# Autodesk Inventor assembly: MotionBaseGeneric
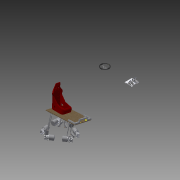
[picture p0: Inventor's stored thumbnail of the model, 180x180]
Saved by Autodesk Inventor 2015 SP1 (Build 190203100, 203)
## iProperties
Created: 2016-02-02
Part Number: MotionBaseGeneric
Document SubType Name: Assembly
Designer: tuttlem
Author: tuttlem
## Documents named in this file (17)
- C:\Users\jonesdm\Desktop\MotionBase\CAD\MotionBaseCAD\MotionBaseGeneric.iam
- C:\Users\jonesdm\Desktop\MotionBase\CAD\MotionBaseCAD\Platform.ipt
- C:\Users\jonesdm\Desktop\MotionBase\CAD\MotionBaseCAD\BasePlatform.ipt
- C:\Users\jonesdm\Desktop\MotionBase\CAD\MotionBaseCAD\Rod.ipt
- C:\Users\jonesdm\Desktop\MotionBase\CAD\MotionBaseCAD\Rod_MIR.ipt
- C:\Users\jonesdm\Desktop\MotionBase\CAD\MotionBaseCAD\arm.ipt
- C:\Users\jonesdm\Desktop\MotionBase\CAD\MotionBaseCAD\Bearing.ipt
- C:\Users\jonesdm\Desktop\MotionBase\CAD\MotionBaseCAD\siege.ipt
- C:\Users\jonesdm\Desktop\MotionBase\CAD\MotionBaseCAD\Sparco Volante wheel.ipt
- C:\Users\jonesdm\Desktop\MotionBase\CAD\MotionBaseCAD\TopPlatform.ipt
- C:\Users\jonesdm\Documents\Inventor\00 - Pedalier CSP V2.iam
- C:\Users\jonesdm\Desktop\MotionBase\CAD\MotionBaseCAD\Side Rail.ipt
- C:\Users\jonesdm\Desktop\MotionBase\CAD\MotionBaseCAD\Front Rail.ipt
- C:\Users\jonesdm\Desktop\MotionBase\CAD\MotionBaseCAD\Imported Components\WGA-50M-080-H1\WGA-50M-080-H1.ipt
- C:\Users\jonesdm\Documents\Motor4.ipt
- C:\Users\jonesdm\Desktop\MotionBase\CAD\MotionBaseCAD\GearShaft.ipt
- C:\Users\jonesdm\Desktop\MotionBase\CAD\MotionBaseCAD\Triangle.ipt
## Components (53 placed, 16 different names)
1. Platform:1 — Insert:3, Insert:5, Mate:1, Flush:7, Mate:2, Flush:8, Mate:3, Mate:4, Mate:5, Flush:9, Wood To Metal, Wood To Back, Mate:66
2. seat — Seat To Wood, Seat To Back, Seat Centered, Angle:9, Mate:72
3. Sparco Volante wheel:1
4. TopPlatform:1 — Wood To Metal, Wood To Back, Angle:8, Seat To Left, Seat To Wood, Seat To Back, Seat Centered, Mate:75, Mate:76, Flush:24, Flush:25, Flush:26, Flush:27, Mate:77, Flush:29, Flush:30, Mate:78, Flush:31, Flush:32
5. Side Rail:1 — Mate:75, Flush:24, Flush:26
6. Side Rail:2 — Mate:76, Flush:25, Flush:27
7. Front Rail:1 — Mate:77, Flush:29, Flush:30
8. Front Rail:2 — Mate:78, Flush:31, Flush:32
9. 00 - Pedalier CSP V2:2 [sub-assembly]
10. GearShaft:2 — Mate:109, Flush:40, Flush:45, Mate:148, Mate:149, Flush:55
11. GearShaft:4 — Mate:111, Flush:42, Flush:45, Mate:146, Mate:147, Flush:54
12. BasePlatform:2
13. GearShaft:8 — Mate:152, Mate:153, Flush:57
14. GearShaft:9 — Mate:154, Mate:155, Flush:58
15. GearShaft:10 — Mate:156, Mate:157, Flush:59
16. GearShaft:11 — Mate:150, Mate:151, Flush:56
17. Triangle:1 — Angle:18, Mate:137, Mate:138, Mate:139, Mate:140, Mate:141, Mate:142
18. Motor4:11 — Flush:52, Mate:129, Angle:16, Angle:17, Symmetry:3
19. Motor4:10 — Flush:52, Symmetry:3
20. Motor4:9 — Flush:53, Mate:130, Angle:16, Symmetry:2
21. Motor4:8 — Flush:53, Symmetry:2
22. Motor4:7 — Mate:96, Angle:17, Symmetry:4
23. Motor4:1 — Mate:79, Angle:10, Mate:80, Mate:91, Symmetry:4
24. Rod_MIR:1 — Flush:1, Tangent:1, Mate:100, Mate:101
25. Rod_MIR:2 — Mate:98, Mate:99
26. Rod_MIR:3 — Mate:28
27. Rod_MIR:4 — Mate:29
28. Rod_MIR:5 — Mate:97
29. Rod_MIR:6 — Mate:32
30. Rod:1 — Flush:1, Tangent:1, Insert:3
31. Rod:2 — Insert:5
32. Rod:3 — Mate:1, Flush:7
33. Rod:4 — Mate:2, Flush:8
34. Rod:5 — Mate:3, Mate:4
35. Rod:6 — Mate:5, Flush:9
36. arm:1 — Mate:146, Mate:147, Flush:54, Mate:162, Flush:64
37. arm:8 — Mate:156, Mate:157, Flush:59, Mate:159, Flush:61
38. arm:9 — Mate:150, Mate:151, Flush:56, Mate:160, Flush:62
39. arm:10 — Mate:154, Mate:155, Flush:58, Mate:158, Flush:60
40. arm:11 — Mate:148, Mate:149, Flush:55, Mate:161, Flush:63
41. arm:12 — Mate:152, Mate:153, Flush:57, Mate:163, Flush:65
42. Bearing:2 — Mate:100, Mate:101, Mate:162, Flush:64
43. Bearing:3 — Mate:97, Mate:159, Flush:61
44. Bearing:4 — Mate:32, Mate:158, Flush:60
45. Bearing:5 — Mate:29, Mate:161, Flush:63
46. Bearing:6 — Mate:28, Mate:160, Flush:62
47. Bearing:1 — Mate:98, Mate:99, Mate:163, Flush:65
48. WGA-50M-080-H1:8 — Mate:136
49. WGA-50M-080-H1:9 — Mate:135
50. WGA-50M-080-H1:10 — Mate:134
51. WGA-50M-080-H1:11 — Mate:133
52. WGA-50M-080-H1:1 — Mate:79, Angle:10, Mate:80, Mate:109, Flush:40, Mate:114, Mate:132
53. WGA-50M-080-H1:7 — Mate:111, Flush:42, Mate:114, Mate:131
## Relationships (147: Mate 80, Flush 44, Angle 12, Tangent 6, Symmetry 3, Insert 2)
- Flush:1: Rod_MIR:1 ↔ Rod:1
- Tangent:1: Rod_MIR:1 ↔ Rod:1
- [Flush]: Rod_MIR:2 ↔ Rod:2
- [Tangent]: Rod_MIR:2 ↔ Rod:2
- Insert:3: Platform:1 ↔ Rod:1
- Insert:5: Platform:1 ↔ Rod:2
- [Flush]: Rod_MIR:3 ↔ Rod:3
- [Tangent]: Rod_MIR:3 ↔ Rod:3
- [Flush]: Rod_MIR:4 ↔ Rod:4
- [Tangent]: Rod_MIR:4 ↔ Rod:4
- [Flush]: Rod_MIR:5 ↔ Rod:5
- [Tangent]: Rod_MIR:5 ↔ Rod:5
- [Flush]: Rod_MIR:6 ↔ Rod:6
- [Tangent]: Rod_MIR:6 ↔ Rod:6
- Mate:1: Platform:1 ↔ Rod:3
- Flush:7: Platform:1 ↔ Rod:3
- Mate:2: Platform:1 ↔ Rod:4
- Flush:8: Platform:1 ↔ Rod:4
- Mate:3: Platform:1 ↔ Rod:5
- Mate:4: Platform:1 ↔ Rod:5
- Mate:5: Platform:1 ↔ Rod:6
- Flush:9: Platform:1 ↔ Rod:6
- Flush:10 (25.4 mm)
- Mate:28: Rod_MIR:3 ↔ Bearing:6
- Mate:29: Rod_MIR:4 ↔ Bearing:5
- Mate:32: Rod_MIR:6 ↔ Bearing:4
- Angle:7 (0 deg)
- Wood To Metal [Mate]: Platform:1 ↔ TopPlatform:1
- Wood To Back [Flush] (-101.6 mm): Platform:1 ↔ TopPlatform:1
- Mate:66: Platform:1
- Angle:8 (0 deg): TopPlatform:1
- Seat To Left [Flush] (-101.6 mm): TopPlatform:1
- Seat To Wood [Mate]: seat ↔ TopPlatform:1
- Seat To Back [Flush] (-76.2 mm): seat ↔ TopPlatform:1
- Seat Centered [Mate]: seat ↔ TopPlatform:1
- Angle:9 (0 deg): seat
- Mate:72: seat
- Mate:75: TopPlatform:1 ↔ Side Rail:1
- Mate:76: TopPlatform:1 ↔ Side Rail:2
- Flush:24: TopPlatform:1 ↔ Side Rail:1
- Flush:25: TopPlatform:1 ↔ Side Rail:2
- Flush:26: TopPlatform:1 ↔ Side Rail:1
- Flush:27: TopPlatform:1 ↔ Side Rail:2
- Mate:77: TopPlatform:1 ↔ Front Rail:1
- Flush:29: TopPlatform:1 ↔ Front Rail:1
- Flush:30: TopPlatform:1 ↔ Front Rail:1
- Mate:78: TopPlatform:1 ↔ Front Rail:2
- Flush:31: TopPlatform:1 ↔ Front Rail:2
- Flush:32: TopPlatform:1 ↔ Front Rail:2
- Mate:79: Motor4:1 ↔ WGA-50M-080-H1:1
- Angle:10 (180 deg): Motor4:1 ↔ WGA-50M-080-H1:1
- Mate:80: Motor4:1 ↔ WGA-50M-080-H1:1
- [Mate]: Motor4:7 ↔ WGA-50M-080-H1:7
- [Angle] (180 deg): Motor4:7 ↔ WGA-50M-080-H1:7
- [Mate]: Motor4:7 ↔ WGA-50M-080-H1:7
- Mate:91: Motor4:1
- Mate:96: Motor4:7
- Mate:97: Rod_MIR:5 ↔ Bearing:3
- Mate:98: Rod_MIR:2 ↔ Bearing:1
- Mate:99: Rod_MIR:2 ↔ Bearing:1
- Mate:100: Rod_MIR:1 ↔ Bearing:2
- Mate:101: Rod_MIR:1 ↔ Bearing:2
- Mate:109: GearShaft:2 ↔ WGA-50M-080-H1:1
- Flush:40 (-114.3 mm): GearShaft:2 ↔ WGA-50M-080-H1:1
- Mate:111: GearShaft:4 ↔ WGA-50M-080-H1:7
- Flush:42 (-114.3 mm): GearShaft:4 ↔ WGA-50M-080-H1:7
- Flush:45: GearShaft:2 ↔ GearShaft:4
- Mate:114 (812.8 mm): WGA-50M-080-H1:1 ↔ WGA-50M-080-H1:7
- [Mate]: Motor4:8 ↔ WGA-50M-080-H1:8
- [Angle] (180 deg): Motor4:8 ↔ WGA-50M-080-H1:8
- [Mate]: Motor4:8 ↔ WGA-50M-080-H1:8
- [Mate]: Motor4:9 ↔ WGA-50M-080-H1:9
- [Angle] (180 deg): Motor4:9 ↔ WGA-50M-080-H1:9
- [Mate]: Motor4:9 ↔ WGA-50M-080-H1:9
- [Mate]: GearShaft:8 ↔ WGA-50M-080-H1:8
- [Flush] (-114.3 mm): GearShaft:8 ↔ WGA-50M-080-H1:8
- [Mate]: GearShaft:9 ↔ WGA-50M-080-H1:9
- [Flush] (-114.3 mm): GearShaft:9 ↔ WGA-50M-080-H1:9
- [Flush]: GearShaft:8 ↔ GearShaft:9
- [Mate] (812.8 mm): WGA-50M-080-H1:8 ↔ WGA-50M-080-H1:9
- [Mate]: Motor4:10 ↔ WGA-50M-080-H1:10
- [Angle] (180 deg): Motor4:10 ↔ WGA-50M-080-H1:10
- [Mate]: Motor4:10 ↔ WGA-50M-080-H1:10
- [Mate]: Motor4:11 ↔ WGA-50M-080-H1:11
- [Angle] (180 deg): Motor4:11 ↔ WGA-50M-080-H1:11
- [Mate]: Motor4:11 ↔ WGA-50M-080-H1:11
- [Mate]: GearShaft:10 ↔ WGA-50M-080-H1:10
- [Flush] (-114.3 mm): GearShaft:10 ↔ WGA-50M-080-H1:10
- [Mate]: GearShaft:11 ↔ WGA-50M-080-H1:11
- [Flush] (-114.3 mm): GearShaft:11 ↔ WGA-50M-080-H1:11
- [Flush]: GearShaft:10 ↔ GearShaft:11
- [Mate] (812.8 mm): WGA-50M-080-H1:10 ↔ WGA-50M-080-H1:11
- Flush:52: Motor4:11 ↔ Motor4:10
- Flush:53: Motor4:9 ↔ Motor4:8
- Mate:129: Motor4:11
- Mate:130: Motor4:9
- Mate:131: WGA-50M-080-H1:7
- Mate:132: WGA-50M-080-H1:1
- Mate:133: WGA-50M-080-H1:11
- Mate:134: WGA-50M-080-H1:10
- Mate:135: WGA-50M-080-H1:9
- Mate:136: WGA-50M-080-H1:8
- Angle:16 (120 deg): Motor4:11 ↔ Motor4:9
- Angle:17 (240 deg): Motor4:11 ↔ Motor4:7
- Symmetry:2: Motor4:9 ↔ Motor4:8
- Symmetry:3: Motor4:11 ↔ Motor4:10
- Symmetry:4: Motor4:7 ↔ Motor4:1
- Angle:18 (0 deg): Triangle:1
- Mate:137: Triangle:1
- Mate:138: Triangle:1
- Mate:139: Triangle:1
- Mate:140: Triangle:1
- Mate:141: Triangle:1
- Mate:142: Triangle:1
- Mate:143 (-762 mm)
- Mate:144 (-762 mm)
- Mate:145 (762 mm)
- Mate:146: GearShaft:4 ↔ arm:1
- Mate:147: GearShaft:4 ↔ arm:1
- Flush:54: GearShaft:4 ↔ arm:1
- Mate:148: GearShaft:2 ↔ arm:11
- Mate:149: GearShaft:2 ↔ arm:11
- Flush:55: GearShaft:2 ↔ arm:11
- Mate:150: GearShaft:11 ↔ arm:9
- Mate:151: GearShaft:11 ↔ arm:9
- Flush:56: GearShaft:11 ↔ arm:9
- Mate:152: GearShaft:8 ↔ arm:12
- Mate:153: GearShaft:8 ↔ arm:12
- Flush:57: GearShaft:8 ↔ arm:12
- Mate:154: GearShaft:9 ↔ arm:10
- Mate:155: GearShaft:9 ↔ arm:10
- Flush:58: GearShaft:9 ↔ arm:10
- Mate:156: GearShaft:10 ↔ arm:8
- Mate:157: GearShaft:10 ↔ arm:8
- Flush:59: GearShaft:10 ↔ arm:8
- Mate:158: arm:10 ↔ Bearing:4
- Mate:159: arm:8 ↔ Bearing:3
- Flush:60: arm:10 ↔ Bearing:4
- Flush:61: arm:8 ↔ Bearing:3
- Mate:160: arm:9 ↔ Bearing:6
- Flush:62: arm:9 ↔ Bearing:6
- Mate:161: arm:11 ↔ Bearing:5
- Flush:63: arm:11 ↔ Bearing:5
- Mate:162: arm:1 ↔ Bearing:2
- Flush:64: arm:1 ↔ Bearing:2
- Mate:163: arm:12 ↔ Bearing:1
- Flush:65: arm:12 ↔ Bearing:1
## Named parameters: d2_d1 = 0 mm, d3_d0 = 0 mm, d18_d1 = 0 mm, d21_d0 = 0 mm, d22_d1 = 0 mm, d25_d0 = 0 mm, d26_d1 = 0 mm, d29_d0 = 0 mm, d30_d1 = 0 mm, d33_d0 = 0 mm, d173_d169 = 0 mm, d174_d171 = 180 deg, d175_d172 = 0 mm, GearShaftL = 152.4 mm, d229_GearShaftL = 152.4 mm, d230_d216 = 0 mm, d231_d217 = -114.3 mm, d232_d220 = 0 mm, d233_d221 = -114.3 mm, d234_d226 = 0 mm, d235_d228 = 812.8 mm, d236_d169 = 0 mm, d237_d171 = 180 deg, d238_d172 = 0 mm, d239_d173_d169 = 0 mm, d240_d174_d171 = 180 deg, d241_d175_d172 = 0 mm, d242_GearShaftL = 152.4 mm, d243_d216 = 0 mm, d244_d217 = -114.3 mm, d245_d220 = 0 mm, d246_d221 = -114.3 mm, d247_d226 = 0 mm, d248_d228 = 812.8 mm, d249_d169 = 0 mm, d250_d171 = 180 deg, d251_d172 = 0 mm, d252_d173_d169 = 0 mm, d253_d174_d171 = 180 deg, d254_d175_d172 = 0 mm
